# Autodesk Inventor assembly: Cyclone
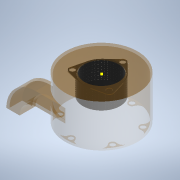
[picture p0: Inventor's stored thumbnail of the model, 180x180]
Saved by Autodesk Inventor 2020 (Build 240168000, 168)
## iProperties
Created: 2020-03-28
Part Number: Cyclone
Document SubType Name: Assembly
Designer: pengpeng
Author: pengpeng
## Documents named in this file (3)
- E:\MENG Project\Open-AMR-Hardware\Hardware\MCAD\Cyclone\Cyclone.iam
- E:\MENG Project\Open-AMR-Hardware\Hardware\MCAD\DustBin\Dust Bin.ipt
- E:\MENG Project\Open-AMR-Hardware\Hardware\MCAD\DustBin\Filter Bin.ipt
## Components (2 placed, 2 different names)
1. Dust Bin:1 — Mate:1, Mate:2, Flush:1, Mate:3, Mate:4, Mate:5
2. Filter Bin:1 — Mate:3, Mate:4, Mate:5
## Relationships (6: Mate 5, Flush 1)
- Mate:1: Dust Bin:1
- Mate:2: Dust Bin:1
- Flush:1: Dust Bin:1
- Mate:3: Dust Bin:1 ↔ Filter Bin:1
- Mate:4: Dust Bin:1 ↔ Filter Bin:1
- Mate:5: Dust Bin:1 ↔ Filter Bin:1
